# Autodesk Inventor assembly: Assembly_Axiotech_Eypiece
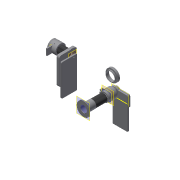
[picture p0: Inventor's stored thumbnail of the model, 180x180]
Saved by Autodesk Inventor 2019 (Build 230136000, 136)
## iProperties
Created: 2019-06-02
Part Number: Assembly_Axiotech_Eypiece
Document SubType Name: Assembly
Designer: diederichbenedict
Author: diederichbenedict
## Documents named in this file (10)
- C:\Users\diederichbenedict\Dropbox\Dokumente\Promotion\PROJECTS\STORMoChip\INVENTOR\Nanoscopy-on-a-cheap\Assembly_Axiotech_Eypiece.iam
- C:\Users\diederichbenedict\Dropbox\Dokumente\Promotion\PROJECTS\STORMoChip\INVENTOR\Nanoscopy-on-a-cheap\00_Zeiss_Axiotech_Eyepiecemount.ipt
- C:\Users\diederichbenedict\Dropbox\Dokumente\Promotion\PROJECTS\STORMoChip\INVENTOR\Nanoscopy-on-a-cheap\10_Zeiss_Axiotech_Eypiecemount_Adapter.ipt
- C:\Users\diederichbenedict\Dropbox\Dokumente\Promotion\PROJECTS\STORMoChip\INVENTOR\Nanoscopy-on-a-cheap\SM30L20-Step.ipt
- C:\Users\diederichbenedict\Dropbox\Dokumente\Promotion\PROJECTS\STORMoChip\INVENTOR\Nanoscopy-on-a-cheap\Assembly_cellphoneadapter.iam
- C:\Users\diederichbenedict\Dropbox\Dokumente\Promotion\PROJECTS\STORMoChip\INVENTOR\Nanoscopy-on-a-cheap\101_Illumination_Adapter_Axiotech_COOLled.ipt
- C:\Users\diederichbenedict\Dropbox\Dokumente\Promotion\PROJECTS\STORMoChip\INVENTOR\Nanoscopy-on-a-cheap\00_Fluegeladapter.ipt
- C:\Users\diederichbenedict\Dropbox\Dokumente\Promotion\PROJECTS\STORMoChip\INVENTOR\Nanoscopy-on-a-cheap\10_Filteslide_25mm.ipt
- C:\Users\diederichbenedict\Dropbox\Dokumente\Promotion\PROJECTS\STORMoChip\INVENTOR\Nanoscopy-on-a-cheap\10_Cellphone_Adapter_30mm_Tube.ipt
- C:\Users\diederichbenedict\Dropbox\Dokumente\Promotion\PROJECTS\STORMoChip\INVENTOR\Nanoscopy-on-a-cheap\100_Huawei_P9.ipt
## Components (10 placed, 9 different names)
1. 00_Zeiss_Axiotech_Eyepiecemount:1 — Flush:1, Flush:2
2. 10_Zeiss_Axiotech_Eypiecemount_Adapter:1 — Flush:1, Flush:2, Insert:1
3. SM30L20-Step:1 — Insert:1, Insert:2
4. Assembly_cellphoneadapter:1 [sub-assembly] — Insert:2
5. 101_Illumination_Adapter_Axiotech_COOLled:1
6. 00_Fluegeladapter:1 — Insert:3, Flush:3, Flush:4
7. SM30L20-Step:2 — Insert:3, Flush:5
8. 10_Filteslide_25mm:1 — Flush:3, Flush:4
9. 10_Cellphone_Adapter_30mm_Tube:1 — Flush:5, Insert:4
10. 100_Huawei_P9:1 — Insert:4
## Relationships (9: Flush 5, Insert 4)
- Flush:1: 00_Zeiss_Axiotech_Eyepiecemount:1 ↔ 10_Zeiss_Axiotech_Eypiecemount_Adapter:1
- Flush:2: 00_Zeiss_Axiotech_Eyepiecemount:1 ↔ 10_Zeiss_Axiotech_Eypiecemount_Adapter:1
- Insert:1: 10_Zeiss_Axiotech_Eypiecemount_Adapter:1 ↔ SM30L20-Step:1
- Insert:2: SM30L20-Step:1 ↔ Assembly_cellphoneadapter:1
- Insert:3: 00_Fluegeladapter:1 ↔ SM30L20-Step:2
- Flush:3: 00_Fluegeladapter:1 ↔ 10_Filteslide_25mm:1
- Flush:4: 00_Fluegeladapter:1 ↔ 10_Filteslide_25mm:1
- Flush:5: SM30L20-Step:2 ↔ 10_Cellphone_Adapter_30mm_Tube:1
- Insert:4: 10_Cellphone_Adapter_30mm_Tube:1 ↔ 100_Huawei_P9:1
